# Autodesk Inventor assembly: Ch-0-01-ChassisFrame
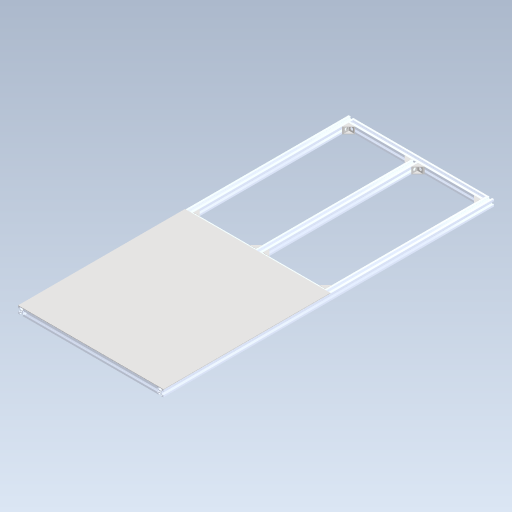
[picture p0: Inventor's stored thumbnail of the model, 512x512]
Saved by Autodesk Inventor 2023 (Build 270158000, 158)
## iProperties
Created: 2023-01-21
Part Number: Ch-0-01-ChassisFrame
Document SubType Name: Assembly
Designer: eplym
Author: eplym
## Documents named in this file (7)
- C:\Users\Dave\Documents\GitHub\BehrendURCMechanical\CAD\Chassis\Ch-0-01-ChassisFrame.iam
- C:\Users\Dave\Documents\GitHub\BehrendURCMechanical\CAD\Chassis\CH-1-01-Longsupport.ipt
- C:\Users\Dave\Documents\GitHub\BehrendURCMechanical\CAD\Chassis\CH-1-01-Shotsupport.ipt
- C:\Users\Dave\Documents\GitHub\BehrendURCMechanical\CAD\Chassis\CH-1-01-middlesupport.ipt
- C:\Users\Dave\Documents\GitHub\BehrendURCMechanical\CAD\Chassis\CH-1-01-support.ipt
- C:\Users\Dave\Documents\GitHub\BehrendURCMechanical\CAD\Chassis\CH-1-01-Sheetmetal.ipt
- C:\Users\Dave\Documents\GitHub\BehrendURCMechanical\CAD\Chassis\CH-1-01-Cornerbracket.ipt
## Components (24 placed, 6 different names)
1. CH-1-01-Longsupport:1 — Mate:1, Flush:3, Flush:4, Mate:19, Mate:20, Mate:33, Mate:35, Flush:11, Flush:12, Flush:13, Flush:14, Flush:15, Flush:23, Flush:24, Flush:27
2. CH-1-01-Longsupport:2 — Mate:2, Mate:3, Flush:1, Flush:2, Mate:7, Flush:6, Flush:9, Mate:12, Mate:27, Mate:29, Mate:43, Flush:26, Flush:29
3. CH-1-01-Shotsupport:1 — Mate:1, Mate:2, Flush:1, Flush:2, Flush:4, Mate:11, Flush:5, Flush:7, Flush:8, Flush:10, Mate:13, Mate:14, Mate:17, Mate:18, Flush:31
4. CH-1-01-Shotsupport:2 — Mate:3, Mate:4, Flush:3, Mate:9, Mate:10, Mate:34, Mate:36, Mate:41, Mate:42, Flush:20, Flush:21, Flush:22, Flush:23, Flush:25
5. CH-1-01-middlesupport:1 — Mate:4, Mate:5, Mate:6, Mate:8, Mate:15, Mate:16, Mate:23, Mate:24, Mate:30, Mate:37, Mate:38, Mate:40, Flush:16, Flush:17, Flush:18, Flush:19, Flush:22, Flush:28
6. CH-1-01-support:1 — Mate:5, Mate:7, Mate:8, Mate:9, Mate:25, Mate:26, Mate:28, Mate:31, Flush:28, Flush:30
7. CH-1-01-support:2 — Mate:6, Mate:10, Mate:21, Mate:22, Mate:32, Mate:39, Flush:14
8. CH-1-01-Sheetmetal:1 — Mate:11, Flush:5, Flush:6, Flush:7, Flush:8, Flush:9, Flush:10
9. CH-1-01-Cornerbracket:1 — Mate:30, Mate:31, Flush:19
10. CH-1-01-Cornerbracket:2 — Mate:32, Mate:33, Flush:15
11. CH-1-01-Cornerbracket:3 — Mate:26, Mate:27, Flush:29
12. CH-1-01-Cornerbracket:4 — Mate:24, Mate:25, Flush:18
13. CH-1-01-Cornerbracket:5 — Mate:28, Mate:29, Flush:30
14. CH-1-01-Cornerbracket:6 — Mate:34, Mate:35, Flush:24
15. CH-1-01-Cornerbracket:7 — Mate:22, Mate:23, Flush:17
16. CH-1-01-Cornerbracket:8 — Mate:20, Mate:21, Flush:13
17. CH-1-01-Cornerbracket:9 — Mate:18, Mate:19, Flush:27
18. CH-1-01-Cornerbracket:10 — Mate:14, Mate:15, Flush:12
19. CH-1-01-Cornerbracket:11 — Mate:16, Mate:17, Flush:11
20. CH-1-01-Cornerbracket:12 — Mate:12, Mate:13, Flush:31
21. CH-1-01-Cornerbracket:13 — Mate:42, Mate:43, Flush:25, Flush:26
22. CH-1-01-Cornerbracket:14 — Mate:38, Mate:39, Flush:16
23. CH-1-01-Cornerbracket:15 — Mate:40, Mate:41, Flush:21
24. CH-1-01-Cornerbracket:16 — Mate:36, Mate:37, Flush:20
## Relationships (74: Mate 43, Flush 31)
- Mate:1: CH-1-01-Longsupport:1 ↔ CH-1-01-Shotsupport:1
- Mate:2: CH-1-01-Longsupport:2 ↔ CH-1-01-Shotsupport:1
- Mate:3: CH-1-01-Longsupport:2 ↔ CH-1-01-Shotsupport:2
- Mate:4: CH-1-01-Shotsupport:2 ↔ CH-1-01-middlesupport:1
- Flush:1: CH-1-01-Longsupport:2 ↔ CH-1-01-Shotsupport:1
- Flush:2: CH-1-01-Longsupport:2 ↔ CH-1-01-Shotsupport:1
- Flush:3: CH-1-01-Longsupport:1 ↔ CH-1-01-Shotsupport:2
- Flush:4: CH-1-01-Longsupport:1 ↔ CH-1-01-Shotsupport:1
- Mate:5: CH-1-01-middlesupport:1 ↔ CH-1-01-support:1
- Mate:6: CH-1-01-middlesupport:1 ↔ CH-1-01-support:2
- Mate:7: CH-1-01-Longsupport:2 ↔ CH-1-01-support:1
- Mate:8: CH-1-01-middlesupport:1 ↔ CH-1-01-support:1
- Mate:9 (470 mm): CH-1-01-Shotsupport:2 ↔ CH-1-01-support:1
- Mate:10 (470 mm): CH-1-01-Shotsupport:2 ↔ CH-1-01-support:2
- Mate:11: CH-1-01-Shotsupport:1 ↔ CH-1-01-Sheetmetal:1
- Flush:5: CH-1-01-Shotsupport:1 ↔ CH-1-01-Sheetmetal:1
- Flush:6: CH-1-01-Longsupport:2 ↔ CH-1-01-Sheetmetal:1
- Flush:7: CH-1-01-Shotsupport:1 ↔ CH-1-01-Sheetmetal:1
- Flush:8: CH-1-01-Shotsupport:1 ↔ CH-1-01-Sheetmetal:1
- Flush:9: CH-1-01-Longsupport:2 ↔ CH-1-01-Sheetmetal:1
- Flush:10: CH-1-01-Shotsupport:1 ↔ CH-1-01-Sheetmetal:1
- Mate:12: CH-1-01-Longsupport:2 ↔ CH-1-01-Cornerbracket:12
- Mate:13: CH-1-01-Shotsupport:1 ↔ CH-1-01-Cornerbracket:12
- Mate:14: CH-1-01-Shotsupport:1 ↔ CH-1-01-Cornerbracket:10
- Mate:15: CH-1-01-middlesupport:1 ↔ CH-1-01-Cornerbracket:10
- Mate:16: CH-1-01-middlesupport:1 ↔ CH-1-01-Cornerbracket:11
- Mate:17: CH-1-01-Shotsupport:1 ↔ CH-1-01-Cornerbracket:11
- Mate:18: CH-1-01-Shotsupport:1 ↔ CH-1-01-Cornerbracket:9
- Mate:19: CH-1-01-Longsupport:1 ↔ CH-1-01-Cornerbracket:9
- Mate:20: CH-1-01-Longsupport:1 ↔ CH-1-01-Cornerbracket:8
- Mate:21: CH-1-01-support:2 ↔ CH-1-01-Cornerbracket:8
- Mate:22: CH-1-01-support:2 ↔ CH-1-01-Cornerbracket:7
- Mate:23: CH-1-01-middlesupport:1 ↔ CH-1-01-Cornerbracket:7
- Mate:24: CH-1-01-middlesupport:1 ↔ CH-1-01-Cornerbracket:4
- Mate:25: CH-1-01-support:1 ↔ CH-1-01-Cornerbracket:4
- Mate:26: CH-1-01-support:1 ↔ CH-1-01-Cornerbracket:3
- Mate:27: CH-1-01-Longsupport:2 ↔ CH-1-01-Cornerbracket:3
- Mate:28: CH-1-01-support:1 ↔ CH-1-01-Cornerbracket:5
- Mate:29: CH-1-01-Longsupport:2 ↔ CH-1-01-Cornerbracket:5
- Mate:30: CH-1-01-middlesupport:1 ↔ CH-1-01-Cornerbracket:1
- Mate:31: CH-1-01-support:1 ↔ CH-1-01-Cornerbracket:1
- Mate:32: CH-1-01-support:2 ↔ CH-1-01-Cornerbracket:2
- Mate:33: CH-1-01-Longsupport:1 ↔ CH-1-01-Cornerbracket:2
- Mate:34: CH-1-01-Shotsupport:2 ↔ CH-1-01-Cornerbracket:6
- Mate:35: CH-1-01-Longsupport:1 ↔ CH-1-01-Cornerbracket:6
- Mate:36: CH-1-01-Shotsupport:2 ↔ CH-1-01-Cornerbracket:16
- Mate:37: CH-1-01-middlesupport:1 ↔ CH-1-01-Cornerbracket:16
- Mate:38: CH-1-01-middlesupport:1 ↔ CH-1-01-Cornerbracket:14
- Mate:39: CH-1-01-support:2 ↔ CH-1-01-Cornerbracket:14
- Mate:40: CH-1-01-middlesupport:1 ↔ CH-1-01-Cornerbracket:15
- Mate:41: CH-1-01-Shotsupport:2 ↔ CH-1-01-Cornerbracket:15
- Mate:42: CH-1-01-Shotsupport:2 ↔ CH-1-01-Cornerbracket:13
- Mate:43: CH-1-01-Longsupport:2 ↔ CH-1-01-Cornerbracket:13
- Flush:11: CH-1-01-Longsupport:1 ↔ CH-1-01-Cornerbracket:11
- Flush:12: CH-1-01-Longsupport:1 ↔ CH-1-01-Cornerbracket:10
- Flush:13: CH-1-01-Longsupport:1 ↔ CH-1-01-Cornerbracket:8
- Flush:14: CH-1-01-Longsupport:1 ↔ CH-1-01-support:2
- Flush:15: CH-1-01-Longsupport:1 ↔ CH-1-01-Cornerbracket:2
- Flush:16: CH-1-01-middlesupport:1 ↔ CH-1-01-Cornerbracket:14
- Flush:17: CH-1-01-middlesupport:1 ↔ CH-1-01-Cornerbracket:7
- Flush:18: CH-1-01-middlesupport:1 ↔ CH-1-01-Cornerbracket:4
- Flush:19: CH-1-01-middlesupport:1 ↔ CH-1-01-Cornerbracket:1
- Flush:20: CH-1-01-Shotsupport:2 ↔ CH-1-01-Cornerbracket:16
- Flush:21: CH-1-01-Shotsupport:2 ↔ CH-1-01-Cornerbracket:15
- Flush:22: CH-1-01-Shotsupport:2 ↔ CH-1-01-middlesupport:1
- Flush:23: CH-1-01-Longsupport:1 ↔ CH-1-01-Shotsupport:2
- Flush:24: CH-1-01-Longsupport:1 ↔ CH-1-01-Cornerbracket:6
- Flush:25: CH-1-01-Shotsupport:2 ↔ CH-1-01-Cornerbracket:13
- Flush:26: CH-1-01-Longsupport:2 ↔ CH-1-01-Cornerbracket:13
- Flush:27: CH-1-01-Longsupport:1 ↔ CH-1-01-Cornerbracket:9
- Flush:28: CH-1-01-middlesupport:1 ↔ CH-1-01-support:1
- Flush:29: CH-1-01-Longsupport:2 ↔ CH-1-01-Cornerbracket:3
- Flush:30: CH-1-01-support:1 ↔ CH-1-01-Cornerbracket:5
- Flush:31: CH-1-01-Shotsupport:1 ↔ CH-1-01-Cornerbracket:12
